# Autodesk Inventor assembly: CuboidTopFrame
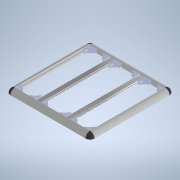
[picture p0: Inventor's stored thumbnail of the model, 180x180]
Saved by Autodesk Inventor 2021 (Build 250183000, 183)
## iProperties
Created: 2020-11-05
Part Number: CuboidTopFrame
Document SubType Name: Assembly
Designer: gisen
Author: gisen
## Documents named in this file (5)
- D:\GitProjects\CAD-Data\CuboidAccessories\CuboidTopFrame\CuboidTopFrame.iam
- D:\GitProjects\CAD-Data\GeneralComponentsTemplate\Fittings\BasicFrameBracket.ipt
- D:\GitProjects\CAD-Data\GeneralComponentsTemplate\Fittings\BasicFrameCornerJoint.ipt
- D:\GitProjects\CAD-Data\CuboidAccessories\CuboidTopFrame\BasicFrameRound330.ipt
- D:\GitProjects\CAD-Data\CuboidAccessories\CuboidTopFrame\BasicFrameLight330.ipt
## Components (22 placed, 4 different names)
1. BasicFrameBracket:1 — メイト:11, メイト:12, メイト:20
2. BasicFrameBracket:2 — メイト:13, メイト:14, メイト:17
3. BasicFrameBracket:3 — メイト:9, メイト:10, メイト:19
4. BasicFrameBracket:4 — メイト:15, メイト:16, メイト:18
5. BasicFrameCornerJoint:1 — メイト:1, フラッシュ:1, フラッシュ:2, メイト:4, フラッシュ:8, フラッシュ:9
6. BasicFrameCornerJoint:2 — メイト:7, メイト:8, フラッシュ:14
7. BasicFrameCornerJoint:3 — メイト:5, フラッシュ:10, フラッシュ:11, メイト:6, フラッシュ:12, フラッシュ:13
8. BasicFrameCornerJoint:4 — フラッシュ:3, メイト:2, フラッシュ:4, メイト:3, フラッシュ:6, フラッシュ:7
9. BasicFrameRound330:1 — メイト:1, フラッシュ:1, フラッシュ:2, フラッシュ:3, メイト:2, フラッシュ:4, メイト:12, メイト:14, フラッシュ:15, 対称度:1, メイト:26
10. BasicFrameRound330:2 — メイト:4, フラッシュ:6, フラッシュ:7, メイト:8, メイト:10, メイト:11, メイト:23, メイト:24, メイト:27, メイト:34, メイト:43, メイト:44, メイト:49, メイト:50, 対称度:2
11. BasicFrameRound330:3 — メイト:6, フラッシュ:12, フラッシュ:13, メイト:7, フラッシュ:14, メイト:9, メイト:15, 対称度:1
12. BasicFrameRound330:4 — メイト:3, フラッシュ:8, フラッシュ:9, メイト:5, フラッシュ:10, フラッシュ:11, メイト:13, メイト:16, フラッシュ:16, フラッシュ:17, メイト:31, メイト:36, メイト:40, メイト:41, メイト:45, メイト:47, 対称度:2
13. BasicFrameLight330:1 — メイト:23, フラッシュ:16, メイト:25, メイト:26, メイト:28, メイト:29, メイト:30, メイト:32, メイト:46, メイト:48
14. BasicFrameLight330:2 — メイト:24, メイト:25, フラッシュ:17, メイト:33, メイト:35, メイト:37, メイト:38, メイト:39, メイト:42
15. BasicFrameBracket:5 — メイト:45, メイト:46, メイト:47
16. BasicFrameBracket:6 — メイト:27, メイト:28, メイト:29
17. BasicFrameBracket:7 — メイト:48, メイト:49, メイト:50
18. BasicFrameBracket:8 — メイト:30, メイト:31, メイト:32
19. BasicFrameBracket:9 — メイト:33, メイト:34, メイト:35
20. BasicFrameBracket:10 — メイト:42, メイト:43, メイト:44
21. BasicFrameBracket:11 — メイト:36, メイト:37, メイト:38
22. BasicFrameBracket:12 — メイト:39, メイト:40, メイト:41
## Relationships (69: Mate 51, Flush 16, Symmetry 2)
- メイト:1 [Mate]: BasicFrameCornerJoint:1 ↔ BasicFrameRound330:1
- フラッシュ:1 [Flush]: BasicFrameCornerJoint:1 ↔ BasicFrameRound330:1
- フラッシュ:2 [Flush]: BasicFrameCornerJoint:1 ↔ BasicFrameRound330:1
- フラッシュ:3 [Flush]: BasicFrameCornerJoint:4 ↔ BasicFrameRound330:1
- メイト:2 [Mate]: BasicFrameCornerJoint:4 ↔ BasicFrameRound330:1
- フラッシュ:4 [Flush]: BasicFrameCornerJoint:4 ↔ BasicFrameRound330:1
- メイト:3 [Mate]: BasicFrameCornerJoint:4 ↔ BasicFrameRound330:4
- メイト:4 [Mate]: BasicFrameCornerJoint:1 ↔ BasicFrameRound330:2
- フラッシュ:6 [Flush]: BasicFrameCornerJoint:4 ↔ BasicFrameRound330:2
- フラッシュ:7 [Flush]: BasicFrameCornerJoint:4 ↔ BasicFrameRound330:2
- フラッシュ:8 [Flush]: BasicFrameCornerJoint:1 ↔ BasicFrameRound330:4
- フラッシュ:9 [Flush]: BasicFrameCornerJoint:1 ↔ BasicFrameRound330:4
- メイト:5 [Mate]: BasicFrameCornerJoint:3 ↔ BasicFrameRound330:4
- フラッシュ:10 [Flush]: BasicFrameCornerJoint:3 ↔ BasicFrameRound330:4
- フラッシュ:11 [Flush]: BasicFrameCornerJoint:3 ↔ BasicFrameRound330:4
- メイト:6 [Mate]: BasicFrameCornerJoint:3 ↔ BasicFrameRound330:3
- フラッシュ:12 [Flush]: BasicFrameCornerJoint:3 ↔ BasicFrameRound330:3
- フラッシュ:13 [Flush]: BasicFrameCornerJoint:3 ↔ BasicFrameRound330:3
- メイト:7 [Mate]: BasicFrameCornerJoint:2 ↔ BasicFrameRound330:3
- メイト:8 [Mate]: BasicFrameCornerJoint:2 ↔ BasicFrameRound330:2
- フラッシュ:14 [Flush]: BasicFrameCornerJoint:2 ↔ BasicFrameRound330:3
- メイト:9 [Mate]: BasicFrameBracket:3 ↔ BasicFrameRound330:3
- メイト:10 [Mate]: BasicFrameBracket:3 ↔ BasicFrameRound330:2
- メイト:11 [Mate]: BasicFrameBracket:1 ↔ BasicFrameRound330:2
- メイト:12 [Mate]: BasicFrameBracket:1 ↔ BasicFrameRound330:1
- メイト:13 [Mate]: BasicFrameBracket:2 ↔ BasicFrameRound330:4
- メイト:14 [Mate]: BasicFrameBracket:2 ↔ BasicFrameRound330:1
- メイト:15 [Mate]: BasicFrameBracket:4 ↔ BasicFrameRound330:3
- メイト:16 [Mate]: BasicFrameBracket:4 ↔ BasicFrameRound330:4
- フラッシュ:15 [Flush] (-10 mm): BasicFrameRound330:1
- メイト:17 [Mate]: BasicFrameBracket:2
- メイト:18 [Mate]: BasicFrameBracket:4
- メイト:19 [Mate]: BasicFrameBracket:3
- メイト:20 [Mate]: BasicFrameBracket:1
- メイト:21 [Mate]
- 対称度:1 [Symmetry]: BasicFrameRound330:1 ↔ BasicFrameRound330:3
- メイト:22 [Mate]
- メイト:23 [Mate]: BasicFrameRound330:2 ↔ BasicFrameLight330:1
- メイト:24 [Mate]: BasicFrameRound330:2 ↔ BasicFrameLight330:2
- フラッシュ:16 [Flush] (-5 mm): BasicFrameRound330:4 ↔ BasicFrameLight330:1
- メイト:25 [Mate] (110 mm): BasicFrameLight330:1 ↔ BasicFrameLight330:2
- フラッシュ:17 [Flush] (-5 mm): BasicFrameRound330:4 ↔ BasicFrameLight330:2
- メイト:26 [Mate] (90 mm): BasicFrameRound330:1 ↔ BasicFrameLight330:1
- メイト:27 [Mate]: BasicFrameRound330:2 ↔ BasicFrameBracket:6
- メイト:28 [Mate]: BasicFrameLight330:1 ↔ BasicFrameBracket:6
- メイト:29 [Mate] (-5 mm): BasicFrameLight330:1 ↔ BasicFrameBracket:6
- メイト:30 [Mate]: BasicFrameLight330:1 ↔ BasicFrameBracket:8
- メイト:31 [Mate]: BasicFrameRound330:4 ↔ BasicFrameBracket:8
- メイト:32 [Mate] (-5 mm): BasicFrameLight330:1 ↔ BasicFrameBracket:8
- メイト:33 [Mate]: BasicFrameLight330:2 ↔ BasicFrameBracket:9
- メイト:34 [Mate]: BasicFrameRound330:2 ↔ BasicFrameBracket:9
- メイト:35 [Mate] (-5 mm): BasicFrameLight330:2 ↔ BasicFrameBracket:9
- メイト:36 [Mate]: BasicFrameRound330:4 ↔ BasicFrameBracket:11
- メイト:37 [Mate]: BasicFrameLight330:2 ↔ BasicFrameBracket:11
- メイト:38 [Mate] (-5 mm): BasicFrameLight330:2 ↔ BasicFrameBracket:11
- メイト:39 [Mate]: BasicFrameLight330:2 ↔ BasicFrameBracket:12
- メイト:40 [Mate]: BasicFrameRound330:4 ↔ BasicFrameBracket:12
- メイト:41 [Mate] (-10 mm): BasicFrameRound330:4 ↔ BasicFrameBracket:12
- メイト:42 [Mate]: BasicFrameLight330:2 ↔ BasicFrameBracket:10
- メイト:43 [Mate]: BasicFrameRound330:2 ↔ BasicFrameBracket:10
- メイト:44 [Mate] (-10 mm): BasicFrameRound330:2 ↔ BasicFrameBracket:10
- メイト:45 [Mate]: BasicFrameRound330:4 ↔ BasicFrameBracket:5
- メイト:46 [Mate]: BasicFrameLight330:1 ↔ BasicFrameBracket:5
- メイト:47 [Mate] (-10 mm): BasicFrameRound330:4 ↔ BasicFrameBracket:5
- メイト:48 [Mate]: BasicFrameLight330:1 ↔ BasicFrameBracket:7
- メイト:49 [Mate]: BasicFrameRound330:2 ↔ BasicFrameBracket:7
- メイト:50 [Mate] (-10 mm): BasicFrameRound330:2 ↔ BasicFrameBracket:7
- 対称度:2 [Symmetry]: BasicFrameRound330:2 ↔ BasicFrameRound330:4
- メイト:51 [Mate]
